# Autodesk Inventor assembly: DayLightGlow
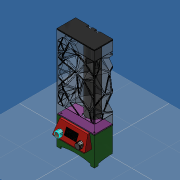
[picture p0: Inventor's stored thumbnail of the model, 180x180]
Saved by Autodesk Inventor 2019 (Build 230136000, 136)
## iProperties
Created: 2019-01-01
Part Number: DayLightGlow
Material: Generisch
Document SubType Name: Assembly
Designer: Stefan
Mass: 2410.56 g
Surface Area: 3145.21 cm^2
Volume: 2063.1 cm^3
Density: 1.16842 g/cm^3
Width: 100,000 mm
Author: Stefan
## Documents named in this file (9)
- C:\Users\User\Documents\Inventor\DayLightGlow\DayLightGlow.iam
- C:\Users\User\Documents\Inventor\DayLightGlow\DayLightGlow_Rod.ipt
- C:\Users\User\Documents\Inventor\DayLightGlow\Crinkle_Lamp\CrinkleLamp_solid_100mm.ipt
- C:\Users\User\Documents\Inventor\DayLightGlow\DayLightGlow_Base.ipt
- C:\Users\User\Documents\Inventor\DayLightGlow\DayLightGlow_SpeakerBase.ipt
- C:\Users\User\Documents\Inventor\DayLightGlow\DayLightGlow_BaseCover.ipt
- C:\Users\User\Documents\Inventor\DayLightGlow\SharpDistanceRanger.ipt
- C:\Users\User\Documents\Inventor\DayLightGlow\Rotary Encoder\rotary encoder_with_knob.iam
- C:\Users\User\Documents\Inventor\DayLightGlow\DayLightGlow_DisplayPanel.iam
## Components (9 placed, 8 different names)
1. DayLightGlow_Rod:1 — Passend:1, Fluchtend:1, Fluchtend:2, Fluchtend:3, Passend:5, Passend:8, Passend:12, Passend:13, Fluchtend:4, Fluchtend:6, Fluchtend:7, Passend:27
2. CrinkleLamp_solid_100mm:1 — Passend:1, Fluchtend:1, Fluchtend:2, Passend:28
3. DayLightGlow_Base:1 — Fluchtend:3, Passend:5, Passend:18, Passend:19, Passend:22, Fluchtend:5, Passend:24, Passend:25, Passend:26, Passend:28
4. DayLightGlow_SpeakerBase:1 — Passend:24, Passend:25, Passend:26
5. DayLightGlow_BaseCover:1 — Passend:8, Passend:12, Passend:13
6. SharpDistanceRanger:1 — Fluchtend:6, Fluchtend:7, Passend:27
7. DayLightGlow_DisplayPanel:2 [sub-assembly] — Fluchtend:4, Passend:16, Passend:17, Passend:22, Fluchtend:5
8. rotary encoder_with_knob:1 [sub-assembly] — Passend:16, Passend:18, Passend:23
9. rotary encoder_with_knob:2 [sub-assembly] — Passend:17, Passend:19, Passend:23
## Relationships (23: Mate 16, Flush 7)
- Passend:1 [Mate]: DayLightGlow_Rod:1 ↔ CrinkleLamp_solid_100mm:1
- Fluchtend:1 [Flush]: DayLightGlow_Rod:1 ↔ CrinkleLamp_solid_100mm:1
- Fluchtend:2 [Flush]: DayLightGlow_Rod:1 ↔ CrinkleLamp_solid_100mm:1
- Fluchtend:3 [Flush]: DayLightGlow_Rod:1 ↔ DayLightGlow_Base:1
- Passend:5 [Mate]: DayLightGlow_Rod:1 ↔ DayLightGlow_Base:1
- Passend:8 [Mate]: DayLightGlow_Rod:1 ↔ DayLightGlow_BaseCover:1
- Passend:12 [Mate]: DayLightGlow_Rod:1 ↔ DayLightGlow_BaseCover:1
- Passend:13 [Mate]: DayLightGlow_Rod:1 ↔ DayLightGlow_BaseCover:1
- Fluchtend:4 [Flush]: DayLightGlow_Rod:1 ↔ DayLightGlow_DisplayPanel:2
- Passend:16 [Mate]: DayLightGlow_DisplayPanel:2 ↔ rotary encoder_with_knob:1
- Passend:17 [Mate]: DayLightGlow_DisplayPanel:2 ↔ rotary encoder_with_knob:2
- Passend:18 [Mate]: DayLightGlow_Base:1 ↔ rotary encoder_with_knob:1
- Passend:19 [Mate]: DayLightGlow_Base:1 ↔ rotary encoder_with_knob:2
- Passend:22 [Mate]: DayLightGlow_Base:1 ↔ DayLightGlow_DisplayPanel:2
- Fluchtend:5 [Flush]: DayLightGlow_Base:1 ↔ DayLightGlow_DisplayPanel:2
- Passend:23 [Mate] (35.27 mm): rotary encoder_with_knob:1 ↔ rotary encoder_with_knob:2
- Passend:24 [Mate]: DayLightGlow_Base:1 ↔ DayLightGlow_SpeakerBase:1
- Passend:25 [Mate]: DayLightGlow_Base:1 ↔ DayLightGlow_SpeakerBase:1
- Passend:26 [Mate]: DayLightGlow_Base:1 ↔ DayLightGlow_SpeakerBase:1
- Fluchtend:6 [Flush]: DayLightGlow_Rod:1 ↔ SharpDistanceRanger:1
- Fluchtend:7 [Flush]: DayLightGlow_Rod:1 ↔ SharpDistanceRanger:1
- Passend:27 [Mate]: DayLightGlow_Rod:1 ↔ SharpDistanceRanger:1
- Passend:28 [Mate]: CrinkleLamp_solid_100mm:1 ↔ DayLightGlow_Base:1
